# Autodesk Inventor assembly: Structure
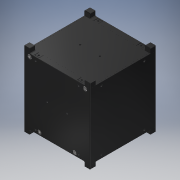
[picture p0: Inventor's stored thumbnail of the model, 180x180]
Saved by Autodesk Inventor 2018 (Build 220112000, 112)
## iProperties
Created: 2018-07-04
Part Number: Structure
Document SubType Name: Assembly
Designer: Bradley
Mass: 606.281 g
Surface Area: 1374.38 cm^2
Volume: 222.571 cm^3
Density: 2.72399 g/cm^3
Author: Bradley
## Documents named in this file (12)
- D:\Users\Bradley\Documents\CougsInSpace\CougSat1-Hardware\CougSat1-Structure\CADModel\Native\Structure.iam
- D:\Users\Bradley\Documents\CougsInSpace\CougSat1-Hardware\CougSat1-Structure\CADModel\Native\Structure_-Y.ipt
- D:\Users\Bradley\Documents\CougsInSpace\CougSat1-Hardware\CougSat1-Structure\CADModel\Native\Structure_+Y.ipt
- D:\Users\Bradley\Documents\CougsInSpace\CougSat1-Hardware\CougSat1-Structure\CADModel\Native\Structure_+Z.ipt
- D:\Users\Bradley\Documents\CougsInSpace\Resources\ComponentModels\Fasteners\Bolt_M3x0.35_12mm_SH.ipt
- D:\Users\Bradley\Documents\CougsInSpace\CougSat1-Hardware\CougSat1-Structure\CADModel\Native\Structure_-Z.ipt
- D:\Users\Bradley\Documents\CougsInSpace\CougSat1-Hardware\CougSat1-Structure\CADModel\Native\Structure_+X.ipt
- D:\Users\Bradley\Documents\CougsInSpace\CougSat1-Hardware\CougSat1-Structure\CADModel\Native\Structure_-X.ipt
- D:\Users\Bradley\Documents\CougsInSpace\Resources\ComponentModels\Hardware\Spring_Separation.ipt
- D:\Users\Bradley\Documents\CougsInSpace\Resources\ComponentModels\Electronics\Switch_Micro-L.iam
- D:\Users\Bradley\Documents\CougsInSpace\Resources\ComponentModels\Hardware\Pin_Headed-2x6mm.ipt
- D:\Users\Bradley\Documents\CougsInSpace\Resources\ComponentModels\Fasteners\Bolt_M1.6x0.35_5mm_SH.ipt
## Components (24 placed, 11 different names)
1. Structure_+X:1 — Mate:1, Flush:6, Flush:7, Insert:16, Insert:19
2. Structure_+Y:1 — Flush:3, Flush:4, Insert:5, Insert:6, Insert:7, Insert:8, Insert:11, Insert:12, Insert:13, Insert:22, Insert:30, Insert:31, Insert:32
3. Structure_+Z:1 — Insert:9, Insert:10, Insert:11, Insert:12, Flush:5, Mate:1, Insert:16, Insert:17, Insert:18
4. Structure_-X:1 — Insert:17, Insert:18, Insert:20
5. Structure_-Y:1 — Flush:1, Flush:2, Insert:1, Insert:2, Insert:3, Insert:4, Insert:9, Insert:10, Insert:14, Insert:15, Insert:21, Flush:10, Insert:25, Insert:26, Insert:27
6. Structure_-Z:1 — Insert:13, Insert:14, Insert:15, Insert:19, Insert:20
7. Switch_Micro-L:1 [sub-assembly] — Flush:10, Insert:23, Insert:24, Insert:26, Insert:27, Tangent:1
8. Switch_Micro-L:2 [sub-assembly] — Insert:30, Insert:31
9. Bolt_M1.6x0.35_5mm_SH:1 — Insert:24
10. Bolt_M1.6x0.35_5mm_SH:2 — Insert:23
11. Bolt_M1.6x0.35_5mm_SH:3
12. Bolt_M1.6x0.35_5mm_SH:4
13. Bolt_M3x0.35_12mm_SH:1 — Insert:1
14. Bolt_M3x0.35_12mm_SH:2 — Insert:2
15. Bolt_M3x0.35_12mm_SH:3 — Insert:3
16. Bolt_M3x0.35_12mm_SH:4 — Insert:4
17. Bolt_M3x0.35_12mm_SH:5 — Insert:5
18. Bolt_M3x0.35_12mm_SH:6 — Insert:7
19. Bolt_M3x0.35_12mm_SH:7 — Insert:6
20. Bolt_M3x0.35_12mm_SH:8 — Insert:8
21. Pin_Headed-2x6mm:1 — Insert:25, Tangent:1
22. Pin_Headed-2x6mm:2 — Insert:32
23. Spring_Separation:1 — Insert:22
24. Spring_Separation:2 — Insert:21
## Relationships (43: Insert 32, Flush 8, Tangent 2, Mate 1)
- Flush:1: Structure_-Y:1
- Flush:2: Structure_-Y:1
- Flush:3: Structure_+Y:1
- Flush:4: Structure_+Y:1
- Insert:1: Structure_-Y:1 ↔ Bolt_M3x0.35_12mm_SH:1
- Insert:2: Structure_-Y:1 ↔ Bolt_M3x0.35_12mm_SH:2
- Insert:3: Structure_-Y:1 ↔ Bolt_M3x0.35_12mm_SH:3
- Insert:4: Structure_-Y:1 ↔ Bolt_M3x0.35_12mm_SH:4
- Insert:5: Structure_+Y:1 ↔ Bolt_M3x0.35_12mm_SH:5
- Insert:6: Structure_+Y:1 ↔ Bolt_M3x0.35_12mm_SH:7
- Insert:7: Structure_+Y:1 ↔ Bolt_M3x0.35_12mm_SH:6
- Insert:8: Structure_+Y:1 ↔ Bolt_M3x0.35_12mm_SH:8
- Insert:9: Structure_+Z:1 ↔ Structure_-Y:1
- Insert:10: Structure_+Z:1 ↔ Structure_-Y:1
- Insert:11: Structure_+Y:1 ↔ Structure_+Z:1
- Insert:12: Structure_+Y:1 ↔ Structure_+Z:1
- Flush:5: Structure_+Z:1
- Insert:13: Structure_+Y:1 ↔ Structure_-Z:1
- Insert:14: Structure_-Y:1 ↔ Structure_-Z:1
- Insert:15: Structure_-Y:1 ↔ Structure_-Z:1
- Mate:1: Structure_+X:1 ↔ Structure_+Z:1
- Flush:6: Structure_+X:1
- Flush:7: Structure_+X:1
- Insert:16: Structure_+X:1 ↔ Structure_+Z:1
- Insert:17: Structure_+Z:1 ↔ Structure_-X:1
- Insert:18: Structure_+Z:1 ↔ Structure_-X:1
- Insert:19: Structure_+X:1 ↔ Structure_-Z:1
- Insert:20: Structure_-X:1 ↔ Structure_-Z:1
- Insert:21: Structure_-Y:1 ↔ Spring_Separation:2
- Insert:22: Structure_+Y:1 ↔ Spring_Separation:1
- Flush:10 (-6.8 mm): Structure_-Y:1 ↔ Switch_Micro-L:1
- Insert:23: Switch_Micro-L:1 ↔ Bolt_M1.6x0.35_5mm_SH:2
- Insert:24: Switch_Micro-L:1 ↔ Bolt_M1.6x0.35_5mm_SH:1
- Insert:25: Structure_-Y:1 ↔ Pin_Headed-2x6mm:1
- Insert:26: Structure_-Y:1 ↔ Switch_Micro-L:1
- Insert:27: Structure_-Y:1 ↔ Switch_Micro-L:1
- Tangent:1: Switch_Micro-L:1 ↔ Pin_Headed-2x6mm:1
- [Insert]: Switch_Micro-L:2 ↔ Bolt_M1.6x0.35_5mm_SH:4
- [Insert]: Switch_Micro-L:2 ↔ Bolt_M1.6x0.35_5mm_SH:3
- [Tangent]: Switch_Micro-L:2 ↔ Pin_Headed-2x6mm:2
- Insert:30: Structure_+Y:1 ↔ Switch_Micro-L:2
- Insert:31: Structure_+Y:1 ↔ Switch_Micro-L:2
- Insert:32: Structure_+Y:1 ↔ Pin_Headed-2x6mm:2
## Named parameters: d49_d48 = 0 mm, d50_d39 = 0 mm, d51_d40 = 0 mm
